# Autodesk Inventor assembly: ASY GNH 021 Dispenser point Frame
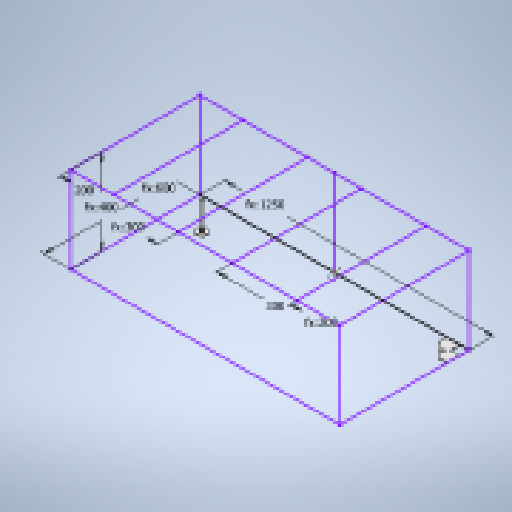
[picture p0: Inventor's stored thumbnail of the model, 512x512]
Saved by Autodesk Inventor 2025.1 (Build 291241020, 241B)
## iProperties
Created: 2025-03-06
Part Number: ASY GNH 021 Dispenser point Frame
Document SubType Name: Assembly
Designer: user
Author: user
## Documents named in this file (5)
- C:\Users\user\YandexDisk-badmisterfox\home pc\Inventor\GNH-Petrodvorec\020 dispenser\020 ASY GNH 010 Dilution point Frame.iam
- C:\Users\user\YandexDisk-badmisterfox\home pc\Inventor\GNH-Petrodvorec\020 dispenser\020 GNH 010 frame.ipt
- C:\Users\user\YandexDisk-badmisterfox\home pc\Inventor\GNH-Petrodvorec\Content Center Files\en-US\ISO 8676(1)\ISO 8676 - M12 x 1.25 x 120DIN EN.ipt
- C:\Users\user\YandexDisk-badmisterfox\home pc\Inventor\GNH-Petrodvorec\GNH 015 leg plate.ipt
- C:\Users\user\YandexDisk-badmisterfox\home pc\Inventor\GNH-Petrodvorec\GNH 015 leg support.ipt
## Components (4 placed, 4 different names)
1. GNH 021 Dispenser Frame1 sketch:1
2. ISO 8676 - M12 x 1.25 x 120:1 — Rigid:2
3. GNH 082 leg plate:1 — Rigid:2
4. GNH 081 leg support:1
## Relationships (1: WeldJoint 1)
- Rigid:2 [WeldJoint]: ISO 8676 - M12 x 1.25 x 120:1 ↔ GNH 082 leg plate:1
